# Autodesk Inventor assembly: Plug P10 femea
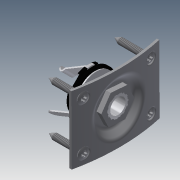
[picture p0: Inventor's stored thumbnail of the model, 180x180]
Saved by Autodesk Inventor 2016 (Build 200138000, 138)
## iProperties
Created: 2018-12-01
Part Number: Plug P10 femea
Document SubType Name: Assembly
Designer: Pedro Mendonça
Author: Pedro Mendonça
## Documents named in this file (5)
- C:\Users\Pedro\Google Drive\Projeto CAD Eng Mecânica\Plug P10 femea.iam
- C:\Users\Pedro\Google Drive\Projeto CAD Eng Mecânica\Plug P10 femea.ipt
- C:\Users\Pedro\Google Drive\Projeto CAD Eng Mecânica\Porca do Plug P10.ipt
- C:\Users\Pedro\Google Drive\Projeto CAD Eng Mecânica\Protetor do Plug P10.ipt
- C:\Users\Pedro\Google Drive\Projeto CAD Eng Mecânica\Parafuso do Plug P10.ipt
## Components (8 placed, 4 different names)
1. Plug P10 femea:1 — Cylindrical:2
2. Porca do Plug P10:1
3. Porca do Plug P10:2 — Cylindrical:2, Cylindrical:3
4. Parafuso do Plug P10:1 — Cylindrical:5
5. Parafuso do Plug P10:2 — Cylindrical:7
6. Parafuso do Plug P10:3 — Cylindrical:6
7. Parafuso do Plug P10:4 — Cylindrical:4
8. Protetor do Plug P10:1 — Cylindrical:3, Cylindrical:4, Cylindrical:5, Cylindrical:6, Cylindrical:7
## Relationships (6: CylindricalJoint 6)
- Cylindrical:2: Plug P10 femea:1 ↔ Porca do Plug P10:2
- Cylindrical:3: Porca do Plug P10:2 ↔ Protetor do Plug P10:1
- Cylindrical:4: Parafuso do Plug P10:4 ↔ Protetor do Plug P10:1
- Cylindrical:5: Parafuso do Plug P10:1 ↔ Protetor do Plug P10:1
- Cylindrical:6: Parafuso do Plug P10:3 ↔ Protetor do Plug P10:1
- Cylindrical:7: Parafuso do Plug P10:2 ↔ Protetor do Plug P10:1
